# Autodesk Inventor assembly: левая лапа - сборка
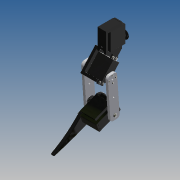
[picture p0: Inventor's stored thumbnail of the model, 180x180]
Saved by Autodesk Inventor 2020 (Build 240168000, 168)
## iProperties
Created: 2019-09-06
Part Number: левая лапа - сборка
Material: Типовые
Document SubType Name: Assembly
Designer: Iliga
Author: Iliga
## Documents named in this file (12)
- F:\GrabCAD\Robot\левая лапа - сборка.iam
- F:\GrabCAD\Robot\двигатель.ipt
- F:\GrabCAD\Robot\kreplenie3.ipt
- F:\GrabCAD\Robot\kreplenie1.ipt
- F:\GrabCAD\Robot\peregorodka.ipt
- F:\GrabCAD\Robot\ship.ipt
- F:\GrabCAD\Robot\kreplenie2.ipt
- F:\GrabCAD\Robot\EN ISO 7045 - M2 x 4 - 4.8 - H(1).ipt
- F:\GrabCAD\Robot\EN ISO 7045 - M4 x 12 - 4.8 - H(1).ipt
- F:\GrabCAD\Robot\EN ISO 7045 - M2 x 10 - 4.8 - H(1).ipt
- F:\GrabCAD\Robot\EN ISO 7045 - M3 x 10 - 4.8 - H(1).ipt
- F:\GrabCAD\Robot\EN ISO 7045 - M2 x 20 - 4.8 - H(1).ipt
## Components (33 placed, 11 different names)
1. двигатель:1 — Совмещение:2, Совмещение:26, Совмещение:27, Совмещение:42, Совмещение:43, Совмещение:44, Совмещение:45, Совмещение:46
2. kreplenie3:1 — Совмещение:2, Совмещение:3, Заподлицо:2, Заподлицо:3, Совмещение:24, Совмещение:26, Совмещение:27
3. kreplenie1:1 — Совмещение:3, Заподлицо:2, Заподлицо:3, Совмещение:4, Совмещение:6, Совмещение:7, Совмещение:21, Совмещение:47, Совмещение:48, Совмещение:49, Совмещение:50
4. двигатель:2 — Совмещение:4, Совмещение:8, Совмещение:9, Совмещение:21, Совмещение:24, Совмещение:51, Совмещение:52, Совмещение:53, Совмещение:54, Совмещение:55, Совмещение:56, Совмещение:57
5. peregorodka:1 — Совмещение:6, Совмещение:7, Совмещение:22, Совмещение:25, Совмещение:33, Совмещение:34, Совмещение:35, Совмещение:36, Совмещение:37, Совмещение:38, Совмещение:39
6. peregorodka:2 — Совмещение:8, Совмещение:9, Совмещение:18, Совмещение:22, Совмещение:28, Совмещение:29, Совмещение:30, Совмещение:31, Совмещение:32, Совмещение:40, Совмещение:41
7. ship:1 — Совмещение:11, Совмещение:12, Совмещение:16, Совмещение:58, Совмещение:59, Совмещение:60, Совмещение:61, Совмещение:62
8. двигатель:3 — Совмещение:11, Совмещение:12, Совмещение:15, Заподлицо:5, Совмещение:16, Совмещение:17, Совмещение:25
9. kreplenie2:1 — Совмещение:15, Заподлицо:5, Совмещение:17, Совмещение:18
10. BS EN ISO 7045 H - метрическая M2 x 4 - 4.8 - H:1 — Заподлицо:6, Заподлицо:8, Совмещение:28
11. BS EN ISO 7045 H - метрическая M2 x 4 - 4.8 - H:2 — Заподлицо:7, Совмещение:29
12. BS EN ISO 7045 H - метрическая M2 x 4 - 4.8 - H:3 — Заподлицо:6, Совмещение:31
13. BS EN ISO 7045 H - метрическая M2 x 4 - 4.8 - H:4 — Заподлицо:7, Заподлицо:8, Совмещение:30, Совмещение:32
14. BS EN ISO 7045 H - метрическая M2 x 4 - 4.8 - H:5 — Заподлицо:13, Заподлицо:15, Совмещение:36, Совмещение:37
15. BS EN ISO 7045 H - метрическая M2 x 4 - 4.8 - H:6 — Заподлицо:14, Заподлицо:15, Совмещение:35
16. BS EN ISO 7045 H - метрическая M2 x 4 - 4.8 - H:7 — Заподлицо:12, Заподлицо:14, Совмещение:34
17. BS EN ISO 7045 H - метрическая M2 x 4 - 4.8 - H:8 — Заподлицо:12, Заподлицо:13, Совмещение:33
18. BS EN ISO 7045 H - метрическая M4 x 12 - 4.8 - H:1 — Совмещение:38, Совмещение:39
19. BS EN ISO 7045 H - метрическая M4 x 12 - 4.8 - H:2 — Совмещение:40, Совмещение:41
20. BS EN ISO 7045 H - метрическая M2 x 10 - 4.8 - H:1 — Заподлицо:16, Заподлицо:17, Совмещение:42
21. BS EN ISO 7045 H - метрическая M2 x 10 - 4.8 - H:2 — Заподлицо:16, Совмещение:43
22. BS EN ISO 7045 H - метрическая M2 x 10 - 4.8 - H:3 — Заподлицо:18, Совмещение:45
23. BS EN ISO 7045 H - метрическая M2 x 10 - 4.8 - H:4 — Заподлицо:17, Заподлицо:18, Совмещение:44, Совмещение:46
24. BS EN ISO 7045 H - метрическая M3 x 10 - 4.8 - H:1 — Совмещение:48, Совмещение:50
25. BS EN ISO 7045 H - метрическая M3 x 10 - 4.8 - H:2 — Совмещение:47, Совмещение:49
26. BS EN ISO 7045 H - метрическая M2 x 10 - 4.8 - H:5 — Совмещение:51, Совмещение:52
27. BS EN ISO 7045 H - метрическая M2 x 10 - 4.8 - H:6 — Совмещение:53, Совмещение:54
28. BS EN ISO 7045 H - метрическая M3 x 10 - 4.8 - H:3 — Заподлицо:19, Совмещение:56
29. BS EN ISO 7045 H - метрическая M3 x 10 - 4.8 - H:4 — Заподлицо:19, Совмещение:55, Совмещение:57
30. BS EN ISO 7045 H - метрическая M2 x 20 - 4.8 - H:1 — Заподлицо:20, Совмещение:59, Совмещение:62
31. BS EN ISO 7045 H - метрическая M2 x 20 - 4.8 - H:2 — Заподлицо:20, Заподлицо:21, Совмещение:58
32. BS EN ISO 7045 H - метрическая M2 x 20 - 4.8 - H:3 — Заподлицо:21, Заподлицо:22, Совмещение:60
33. BS EN ISO 7045 H - метрическая M2 x 20 - 4.8 - H:4 — Заподлицо:22, Совмещение:61
## Relationships (74: Mate 54, Flush 20)
- Совмещение:2 [Mate]: двигатель:1 ↔ kreplenie3:1
- Совмещение:3 [Mate]: kreplenie3:1 ↔ kreplenie1:1
- Заподлицо:2 [Flush]: kreplenie3:1 ↔ kreplenie1:1
- Заподлицо:3 [Flush]: kreplenie3:1 ↔ kreplenie1:1
- Совмещение:4 [Mate]: kreplenie1:1 ↔ двигатель:2
- Совмещение:6 [Mate]: kreplenie1:1 ↔ peregorodka:1
- Совмещение:7 [Mate]: kreplenie1:1 ↔ peregorodka:1
- Совмещение:8 [Mate]: двигатель:2 ↔ peregorodka:2
- Совмещение:9 [Mate]: двигатель:2 ↔ peregorodka:2
- Совмещение:11 [Mate]: ship:1 ↔ двигатель:3
- Совмещение:12 [Mate]: ship:1 ↔ двигатель:3
- Совмещение:15 [Mate]: двигатель:3 ↔ kreplenie2:1
- Заподлицо:5 [Flush]: двигатель:3 ↔ kreplenie2:1
- Совмещение:16 [Mate]: ship:1 ↔ двигатель:3
- Совмещение:17 [Mate]: двигатель:3 ↔ kreplenie2:1
- Совмещение:18 [Mate]: peregorodka:2 ↔ kreplenie2:1
- Совмещение:21 [Mate]: kreplenie1:1 ↔ двигатель:2
- Совмещение:22 [Mate]: peregorodka:1 ↔ peregorodka:2
- Совмещение:24 [Mate]: kreplenie3:1 ↔ двигатель:2
- Совмещение:25 [Mate]: peregorodka:1 ↔ двигатель:3
- Совмещение:26 [Mate]: двигатель:1 ↔ kreplenie3:1
- Совмещение:27 [Mate]: двигатель:1 ↔ kreplenie3:1
- Заподлицо:6 [Flush]: BS EN ISO 7045 H - метрическая M2 x 4 - 4.8 - H:1 ↔ BS EN ISO 7045 H - метрическая M2 x 4 - 4.8 - H:3
- Заподлицо:7 [Flush]: BS EN ISO 7045 H - метрическая M2 x 4 - 4.8 - H:2 ↔ BS EN ISO 7045 H - метрическая M2 x 4 - 4.8 - H:4
- Заподлицо:8 [Flush]: BS EN ISO 7045 H - метрическая M2 x 4 - 4.8 - H:1 ↔ BS EN ISO 7045 H - метрическая M2 x 4 - 4.8 - H:4
- Совмещение:28 [Mate]: peregorodka:2 ↔ BS EN ISO 7045 H - метрическая M2 x 4 - 4.8 - H:1
- Совмещение:29 [Mate]: peregorodka:2 ↔ BS EN ISO 7045 H - метрическая M2 x 4 - 4.8 - H:2
- Совмещение:30 [Mate]: peregorodka:2 ↔ BS EN ISO 7045 H - метрическая M2 x 4 - 4.8 - H:4
- Совмещение:31 [Mate]: peregorodka:2 ↔ BS EN ISO 7045 H - метрическая M2 x 4 - 4.8 - H:3
- Совмещение:32 [Mate]: peregorodka:2 ↔ BS EN ISO 7045 H - метрическая M2 x 4 - 4.8 - H:4
- [Flush]: BS EN ISO 7045 H - метрическая M2 x 4 - 4.8 - H:5 ↔ BS EN ISO 7045 H - метрическая M2 x 4 - 4.8 - H:7
- [Flush]: BS EN ISO 7045 H - метрическая M2 x 4 - 4.8 - H:6 ↔ BS EN ISO 7045 H - метрическая M2 x 4 - 4.8 - H:8
- [Flush]: BS EN ISO 7045 H - метрическая M2 x 4 - 4.8 - H:5 ↔ BS EN ISO 7045 H - метрическая M2 x 4 - 4.8 - H:8
- Заподлицо:12 [Flush]: BS EN ISO 7045 H - метрическая M2 x 4 - 4.8 - H:7 ↔ BS EN ISO 7045 H - метрическая M2 x 4 - 4.8 - H:8
- Заподлицо:13 [Flush]: BS EN ISO 7045 H - метрическая M2 x 4 - 4.8 - H:5 ↔ BS EN ISO 7045 H - метрическая M2 x 4 - 4.8 - H:8
- Заподлицо:14 [Flush]: BS EN ISO 7045 H - метрическая M2 x 4 - 4.8 - H:6 ↔ BS EN ISO 7045 H - метрическая M2 x 4 - 4.8 - H:7
- Заподлицо:15 [Flush]: BS EN ISO 7045 H - метрическая M2 x 4 - 4.8 - H:5 ↔ BS EN ISO 7045 H - метрическая M2 x 4 - 4.8 - H:6
- Совмещение:33 [Mate]: peregorodka:1 ↔ BS EN ISO 7045 H - метрическая M2 x 4 - 4.8 - H:8
- Совмещение:34 [Mate]: peregorodka:1 ↔ BS EN ISO 7045 H - метрическая M2 x 4 - 4.8 - H:7
- Совмещение:35 [Mate]: peregorodka:1 ↔ BS EN ISO 7045 H - метрическая M2 x 4 - 4.8 - H:6
- Совмещение:36 [Mate]: peregorodka:1 ↔ BS EN ISO 7045 H - метрическая M2 x 4 - 4.8 - H:5
- Совмещение:37 [Mate]: peregorodka:1 ↔ BS EN ISO 7045 H - метрическая M2 x 4 - 4.8 - H:5
- Совмещение:38 [Mate]: peregorodka:1 ↔ BS EN ISO 7045 H - метрическая M4 x 12 - 4.8 - H:1
- Совмещение:39 [Mate]: peregorodka:1 ↔ BS EN ISO 7045 H - метрическая M4 x 12 - 4.8 - H:1
- Совмещение:40 [Mate]: peregorodka:2 ↔ BS EN ISO 7045 H - метрическая M4 x 12 - 4.8 - H:2
- Совмещение:41 [Mate]: peregorodka:2 ↔ BS EN ISO 7045 H - метрическая M4 x 12 - 4.8 - H:2
- Заподлицо:16 [Flush]: BS EN ISO 7045 H - метрическая M2 x 10 - 4.8 - H:1 ↔ BS EN ISO 7045 H - метрическая M2 x 10 - 4.8 - H:2
- Заподлицо:17 [Flush]: BS EN ISO 7045 H - метрическая M2 x 10 - 4.8 - H:1 ↔ BS EN ISO 7045 H - метрическая M2 x 10 - 4.8 - H:4
- Заподлицо:18 [Flush]: BS EN ISO 7045 H - метрическая M2 x 10 - 4.8 - H:3 ↔ BS EN ISO 7045 H - метрическая M2 x 10 - 4.8 - H:4
- Совмещение:42 [Mate]: двигатель:1 ↔ BS EN ISO 7045 H - метрическая M2 x 10 - 4.8 - H:1
- Совмещение:43 [Mate]: двигатель:1 ↔ BS EN ISO 7045 H - метрическая M2 x 10 - 4.8 - H:2
- Совмещение:44 [Mate]: двигатель:1 ↔ BS EN ISO 7045 H - метрическая M2 x 10 - 4.8 - H:4
- Совмещение:45 [Mate]: двигатель:1 ↔ BS EN ISO 7045 H - метрическая M2 x 10 - 4.8 - H:3
- Совмещение:46 [Mate]: двигатель:1 ↔ BS EN ISO 7045 H - метрическая M2 x 10 - 4.8 - H:4
- Совмещение:47 [Mate]: kreplenie1:1 ↔ BS EN ISO 7045 H - метрическая M3 x 10 - 4.8 - H:2
- Совмещение:48 [Mate]: kreplenie1:1 ↔ BS EN ISO 7045 H - метрическая M3 x 10 - 4.8 - H:1
- Совмещение:49 [Mate]: kreplenie1:1 ↔ BS EN ISO 7045 H - метрическая M3 x 10 - 4.8 - H:2
- Совмещение:50 [Mate]: kreplenie1:1 ↔ BS EN ISO 7045 H - метрическая M3 x 10 - 4.8 - H:1
- Совмещение:51 [Mate]: двигатель:2 ↔ BS EN ISO 7045 H - метрическая M2 x 10 - 4.8 - H:5
- Совмещение:52 [Mate]: двигатель:2 ↔ BS EN ISO 7045 H - метрическая M2 x 10 - 4.8 - H:5
- Совмещение:53 [Mate]: двигатель:2 ↔ BS EN ISO 7045 H - метрическая M2 x 10 - 4.8 - H:6
- Совмещение:54 [Mate]: двигатель:2 ↔ BS EN ISO 7045 H - метрическая M2 x 10 - 4.8 - H:6
- Заподлицо:19 [Flush]: BS EN ISO 7045 H - метрическая M3 x 10 - 4.8 - H:3 ↔ BS EN ISO 7045 H - метрическая M3 x 10 - 4.8 - H:4
- Совмещение:55 [Mate]: двигатель:2 ↔ BS EN ISO 7045 H - метрическая M3 x 10 - 4.8 - H:4
- Совмещение:56 [Mate]: двигатель:2 ↔ BS EN ISO 7045 H - метрическая M3 x 10 - 4.8 - H:3
- Совмещение:57 [Mate]: двигатель:2 ↔ BS EN ISO 7045 H - метрическая M3 x 10 - 4.8 - H:4
- Заподлицо:20 [Flush]: BS EN ISO 7045 H - метрическая M2 x 20 - 4.8 - H:1 ↔ BS EN ISO 7045 H - метрическая M2 x 20 - 4.8 - H:2
- Заподлицо:21 [Flush]: BS EN ISO 7045 H - метрическая M2 x 20 - 4.8 - H:2 ↔ BS EN ISO 7045 H - метрическая M2 x 20 - 4.8 - H:3
- Заподлицо:22 [Flush]: BS EN ISO 7045 H - метрическая M2 x 20 - 4.8 - H:3 ↔ BS EN ISO 7045 H - метрическая M2 x 20 - 4.8 - H:4
- Совмещение:58 [Mate]: ship:1 ↔ BS EN ISO 7045 H - метрическая M2 x 20 - 4.8 - H:2
- Совмещение:59 [Mate]: ship:1 ↔ BS EN ISO 7045 H - метрическая M2 x 20 - 4.8 - H:1
- Совмещение:60 [Mate]: ship:1 ↔ BS EN ISO 7045 H - метрическая M2 x 20 - 4.8 - H:3
- Совмещение:61 [Mate]: ship:1 ↔ BS EN ISO 7045 H - метрическая M2 x 20 - 4.8 - H:4
- Совмещение:62 [Mate]: ship:1 ↔ BS EN ISO 7045 H - метрическая M2 x 20 - 4.8 - H:1
## Named parameters: d44_d36 = 0 mm, d45_d37 = 0 mm, d46_d38 = 0 mm
